# Autodesk Inventor assembly: testassembly
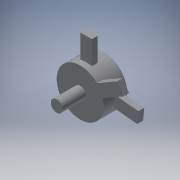
[picture p0: Inventor's stored thumbnail of the model, 180x180]
Saved by Autodesk Inventor 2016 (Build 200138000, 138)
## iProperties
Created: 2015-12-12
Part Number: testassembly
Document SubType Name: Assembly
Designer: Louis
Author: Louis
## Documents named in this file (3)
- C:\Users\Louis\Desktop\testcadstuff\testassembly.iam
- C:\Users\Louis\Desktop\testcadstuff\holder.ipt
- C:\Users\Louis\Desktop\testcadstuff\spinnything.ipt
## Components (4 placed, 2 different names)
1. holder:1 — Mate:1, Mate:2, Mate:4, Mate:6
2. spinnything:1 — Mate:1, Mate:2, Mate:3
3. spinnything:2 — Mate:3, Mate:4, Mate:5
4. spinnything:3 — Mate:5, Mate:6
## Relationships (6: Mate 6)
- Mate:1: holder:1 ↔ spinnything:1
- Mate:2: holder:1 ↔ spinnything:1
- Mate:3: spinnything:1 ↔ spinnything:2
- Mate:4: holder:1 ↔ spinnything:2
- Mate:5: spinnything:2 ↔ spinnything:3
- Mate:6: holder:1 ↔ spinnything:3
